# Autodesk Inventor assembly: x_axis_base_rails
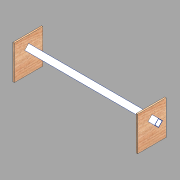
[picture p0: Inventor's stored thumbnail of the model, 180x180]
Saved by Autodesk Inventor 2020 (Build 240168000, 168)
## iProperties
Created: 2021-04-02
Part Number: x_axis_base_rails
Document SubType Name: Assembly
Designer: griss
Mass: 310.202 g
Surface Area: 1422.6 cm^2
Volume: 177.031 cm^3
Density: 1.75225 g/cm^3
Author: griss
## Documents named in this file (9)
- C:\Users\griss\Documents\Inventor\CNC\x_axis\x_axis_base_rails.iam
- C:\Users\griss\Documents\Inventor\CNC\x_axis\x_axis_base_rail.ipt
- C:\Users\griss\Documents\Inventor\CNC\x_axis\x_axis_wood_mount.ipt
- C:\Users\griss\Documents\Inventor\CNC\x_axis\x_axis_base_rails\AIP\FEA\dkbzbftj4.fins
- C:\Users\griss\Documents\Inventor\CNC\x_axis\x_axis_base_rails\AIP\FEA\dkbzbftj4.fsat
- C:\Users\griss\Documents\Inventor\CNC\x_axis\x_axis_base_rails\AIP\FEA\dkbzbftk0.ftes
- C:\Users\griss\Documents\Inventor\CNC\x_axis\x_axis_base_rails\AIP\FEA\dkbzbftk0.fwiz
- C:\Users\griss\Documents\Inventor\CNC\x_axis\x_axis_base_rails\AIP\FEA\dkbzbftkw.fmsh
- C:\Users\griss\Documents\Inventor\CNC\x_axis\x_axis_base_rails\AIP\FEA\dkbzbftkx.fres
## Components (3 placed, 2 different names)
1. x_axis_base_rail:1 — Mate:1, Mate:2, Mate:3, Mate:4, Flush:1, Flush:2
2. x_axis_wood_mount:1 — Mate:1, Mate:2, Flush:2
3. x_axis_wood_mount:2 — Mate:3, Mate:4, Flush:1
## Relationships (6: Mate 4, Flush 2)
- Mate:1: x_axis_base_rail:1 ↔ x_axis_wood_mount:1
- Mate:2: x_axis_base_rail:1 ↔ x_axis_wood_mount:1
- Mate:3: x_axis_base_rail:1 ↔ x_axis_wood_mount:2
- Mate:4: x_axis_base_rail:1 ↔ x_axis_wood_mount:2
- Flush:1 (-29.21 mm): x_axis_base_rail:1 ↔ x_axis_wood_mount:2
- Flush:2 (-25.4 mm): x_axis_base_rail:1 ↔ x_axis_wood_mount:1
## Named parameters: sa_0 = 22241.1
note: some values were not read from the file. Shown as the stored number, unit unknown: "sa_0".
